# Autodesk Inventor assembly: AxisZ
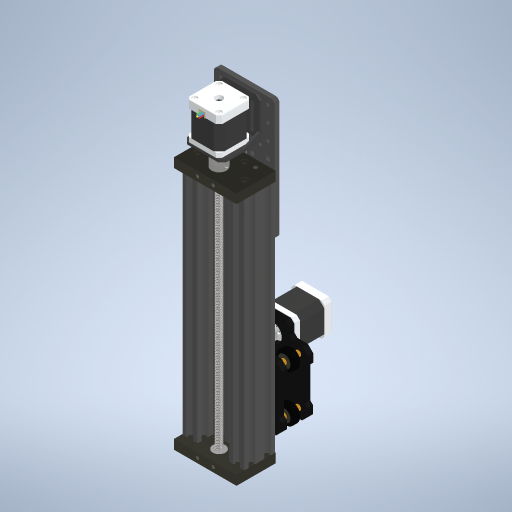
[picture p0: Inventor's stored thumbnail of the model, 512x512]
Saved by Autodesk Inventor 2024.2 (Build 282272000, 272)
## iProperties
Created: 2024-08-27
Part Number: AxisZ
Document SubType Name: Assembly
Designer: Admin
Author: Admin
## Documents named in this file (12)
- C:\Users\Admin\Documents\GitHub\ManipuladorCartesiano\DiseñoMecánico\Assemblies\AxisZ.iam
- C:\Users\Admin\Documents\GitHub\ManipuladorCartesiano\DiseñoMecánico\Axis\AxisZ\Structure\C-Beam4080.ipt
- C:\Users\Admin\Documents\GitHub\ManipuladorCartesiano\DiseñoMecánico\Axis\AxisZ\Structure\C-BeamEnd.ipt
- C:\Users\Admin\Documents\GitHub\ManipuladorCartesiano\DiseñoMecánico\Axis\AxisZ\Structure\Bearing8x16x5.ipt
- C:\Users\Admin\Documents\GitHub\ManipuladorCartesiano\DiseñoMecánico\Axis\AxisZ\Structure\BallScrew.ipt
- C:\Users\Admin\Documents\GitHub\ManipuladorCartesiano\DiseñoMecánico\Assemblies\SlidingHolder.iam
- C:\Users\Admin\Documents\GitHub\ManipuladorCartesiano\DiseñoMecánico\AuxiliarPieces\GantryPlate\C-Beam CNC.ipt
- C:\Users\Admin\Documents\GitHub\ManipuladorCartesiano\DiseñoMecánico\AuxiliarPieces\BracketNEMA17\BracketNEMA17.ipt
- C:\Users\Admin\Documents\GitHub\ManipuladorCartesiano\DiseñoMecánico\AuxiliarPieces\Coupler[6.35-8]\Coupler[6.35-8].ipt
- Coupler[6.35-8].ipt
- C:\Users\Admin\Documents\GitHub\ManipuladorCartesiano\DiseñoMecánico\Motors\NEMA17 [48mm]\NEMA17 [48mm].ipt
- C:\Users\Admin\Documents\GitHub\ManipuladorCartesiano\DiseñoMecánico\AuxiliarPieces\Pulley\GT2_20T\GT2_20T.ipt
## Components (12 placed, 10 different names)
1. SlidingHolder:1 [sub-assembly] — Mate:9, Flush:6, Flush:8, Mate:18, Flush:10
2. C-Beam CNC:1 — Mate:8, Flush:7, Flush:9
3. BracketNEMA17:1 — Mate:12, Mate:13, Mate:14, Mate:15, Flush:9
4. Coupler[6.35-8]:1 — Mate:11, Mate:15, Mate:16, Mate:17
5. NEMA17 [48mm]:1 — Mate:11, Mate:12, Mate:13, Mate:14
6. GT2_20T:1 — Mate:18, Flush:10
7. C-Beam4080:1 — Flush:1, Mate:1, Mate:2, Flush:2, Flush:3, Flush:4, Mate:9
8. C-BeamEnd:2 — Mate:2, Flush:3, Flush:4, Mate:3, Mate:4, Flush:5, Flush:6, Flush:8
9. C-BeamEnd:3 — Flush:1, Mate:1, Flush:2, Mate:5, Mate:6, Mate:7, Mate:8, Mate:16, Mate:17, Flush:7
10. Bearing8x16x5:1 — Mate:3, Mate:4
11. Bearing8x16x5:2 — Mate:5, Mate:6
12. BallScrew:1 — Mate:7, Flush:5
## Relationships (27: Mate 17, Flush 10)
- Flush:1: C-Beam4080:1 ↔ C-BeamEnd:3
- Mate:1: C-Beam4080:1 ↔ C-BeamEnd:3
- Mate:2: C-Beam4080:1 ↔ C-BeamEnd:2
- Flush:2: C-Beam4080:1 ↔ C-BeamEnd:3
- Flush:3: C-Beam4080:1 ↔ C-BeamEnd:2
- Flush:4: C-Beam4080:1 ↔ C-BeamEnd:2
- Mate:3: C-BeamEnd:2 ↔ Bearing8x16x5:1
- Mate:4: C-BeamEnd:2 ↔ Bearing8x16x5:1
- Mate:5: C-BeamEnd:3 ↔ Bearing8x16x5:2
- Mate:6: C-BeamEnd:3 ↔ Bearing8x16x5:2
- Mate:7: C-BeamEnd:3 ↔ BallScrew:1
- Flush:5: C-BeamEnd:2 ↔ BallScrew:1
- Mate:8: C-Beam CNC:1 ↔ C-BeamEnd:3
- Mate:9 (4.9 mm): SlidingHolder:1 ↔ C-Beam4080:1
- Flush:6 (26 mm): SlidingHolder:1 ↔ C-BeamEnd:2
- Mate:11: Coupler[6.35-8]:1 ↔ NEMA17 [48mm]:1
- Mate:12: BracketNEMA17:1 ↔ NEMA17 [48mm]:1
- Mate:13: BracketNEMA17:1 ↔ NEMA17 [48mm]:1
- Mate:14: BracketNEMA17:1 ↔ NEMA17 [48mm]:1
- Mate:15: BracketNEMA17:1 ↔ Coupler[6.35-8]:1
- Mate:16 (1 mm): Coupler[6.35-8]:1 ↔ C-BeamEnd:3
- Mate:17: Coupler[6.35-8]:1 ↔ C-BeamEnd:3
- Flush:7 (1.25 mm): C-Beam CNC:1 ↔ C-BeamEnd:3
- Flush:8 (1 mm): SlidingHolder:1 ↔ C-BeamEnd:2
- Flush:9: C-Beam CNC:1 ↔ BracketNEMA17:1
- Mate:18: SlidingHolder:1 ↔ GT2_20T:1
- Flush:10: SlidingHolder:1 ↔ GT2_20T:1
